# Autodesk Inventor assembly: case
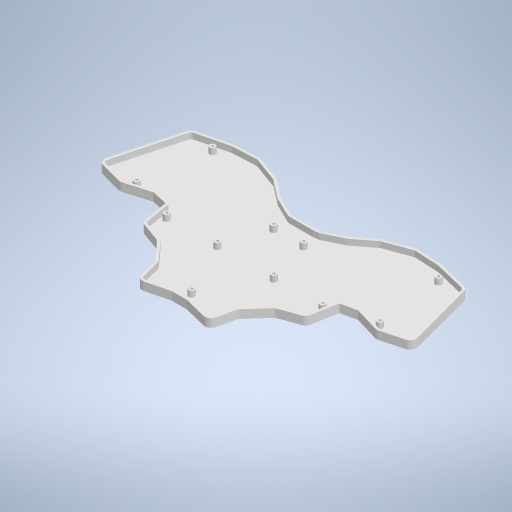
[picture p0: Inventor's stored thumbnail of the model, 512x512]
Saved by Autodesk Inventor 2024 (Build 280153000, 153)
## iProperties
Created: 2024-09-29
Part Number: case
Document SubType Name: Assembly
Designer: nikla
Author: nikla
## Documents named in this file (6)
- C:\Users\nikla\OneDrive\Keyboards\Blavinge\case\1-part\bottom.iam
- C:\Users\nikla\OneDrive\Keyboards\Blavinge\kicad\blavinge\blavinge.iam
- C:\Users\nikla\OneDrive\Keyboards\Blavinge\case\1-part\middle_bottom.ipt
- C:\Users\nikla\OneDrive\Keyboards\Blavinge\case\1-part\left_bottom.ipt
- C:\Users\nikla\OneDrive\Keyboards\Blavinge\case\1-part\left_bottom_MIR.ipt
- C:\Users\nikla\OneDrive\Keyboards\Blavinge\case\1-part\bottom.ipt
## Components (5 placed, 5 different names)
1. blavinge:1 [sub-assembly] — Fluchtend:2, Fluchtend:5, Fluchtend:6
2. middle_bottom:1 — Fluchtend:2, Fluchtend:7
3. left_bottom:1 — Fluchtend:5, Fluchtend:6
4. left_bottom_MIR:1
5. bottom:1 — Fluchtend:7
## Relationships (4: Flush 4)
- Fluchtend:2 [Flush]: blavinge:1 ↔ middle_bottom:1
- Fluchtend:5 [Flush]: blavinge:1 ↔ left_bottom:1
- Fluchtend:6 [Flush]: blavinge:1 ↔ left_bottom:1
- Fluchtend:7 [Flush]: middle_bottom:1 ↔ bottom:1
